# Autodesk Inventor assembly: Assembly1
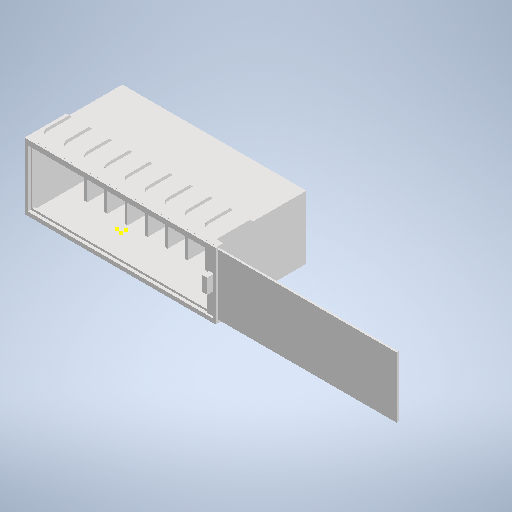
[picture p0: Inventor's stored thumbnail of the model, 512x512]
Saved by Autodesk Inventor 2025.2 (Build 292293000, 293)
## iProperties
Created: 2025-04-07
Part Number: Assembly1
Document SubType Name: Assembly
Designer: LabB305
Author: LabB305
## Documents named in this file (4)
- C:\Users\LabB305\Documents\Modelos\Assembly1.iam
- C:\Users\LabB305\Documents\Modelos\Door.ipt
- C:\Users\LabB305\Documents\Modelos\Front cover.ipt
- C:\Users\LabB305\Documents\Modelos\Storage.ipt
## Components (3 placed, 3 different names)
1. Door:1 — Mate:1
2. Front cover:1 — Rigid:1
3. Storage:1 — Mate:1, Rigid:1
## Relationships (2: Mate 1, WeldJoint 1)
- Mate:1: Door:1 ↔ Storage:1
- Rigid:1 [WeldJoint] (-95.75 mm): Front cover:1 ↔ Storage:1
